# Autodesk Inventor assembly: Arm_Flame_2_8
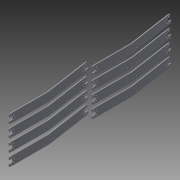
[picture p0: Inventor's stored thumbnail of the model, 180x180]
Saved by Autodesk Inventor 2013 (Build 170138000, 138)
## iProperties
Created: 2014-05-16
Part Number: Arm_Flame_2_8
Document SubType Name: Assembly
Designer: andou
Author: andou
## Documents named in this file (2)
- C:\Users\andou\Documents\Inventor\RoboticsProject\project_4\Robot\Arm\Arm_Flame_2_8.iam
- C:\Users\andou\Documents\Inventor\RoboticsProject\project_4\Robot\Arm\Arm_Link_1.ipt
## Components (8 placed, 1 different names)
1. Arm_Link_1:1
2. Arm_Link_1:2
3. Arm_Link_1:3
4. Arm_Link_1:4
5. Arm_Link_1:5
6. Arm_Link_1:6
7. Arm_Link_1:7
8. Arm_Link_1:8
## Component patterns: (8 elements, first: Arm_Link_1:1)
